# Autodesk Inventor assembly: Sample 1
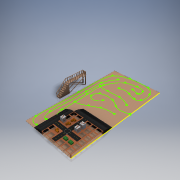
[picture p0: Inventor's stored thumbnail of the model, 180x180]
Saved by Autodesk Inventor 2019 (Build 230136000, 136)
## iProperties
Created: 2020-04-28
Part Number: Sample 1
Document SubType Name: Assembly
Designer: infinity
Author: infinity
## Documents named in this file (12)
- C:\Users\infinity\Documents\GitHub\barc_hardware\Track Sample 1\Sample 1.iam
- C:\Users\infinity\Documents\GitHub\barc_hardware\Track Sample 1\floor_50_100.ipt
- C:\Users\infinity\Documents\GitHub\barc_hardware\Track Sample 1\2ft stand.ipt
- C:\Users\infinity\Documents\GitHub\barc_hardware\Track Sample 1\Ramp 1.ipt
- C:\Users\infinity\Documents\GitHub\barc_hardware\Track Sample 1\driver stand.ipt
- C:\Users\infinity\Documents\GitHub\barc_hardware\Track Sample 1\house_1.ipt
- C:\Users\infinity\Documents\GitHub\barc_hardware\Track Sample 1\building_1.ipt
- C:\Users\infinity\Documents\GitHub\barc_hardware\Track Sample 1\apartment_1.ipt
- C:\Users\infinity\Documents\GitHub\barc_hardware\Track Sample 1\road_empty.ipt
- C:\Users\infinity\Documents\GitHub\barc_hardware\Track Sample 1\intersection_1.ipt
- C:\Users\infinity\Documents\GitHub\barc_hardware\Track Sample 1\black_mid_yellow line.ipt
- C:\Users\infinity\Documents\GitHub\barc_hardware\Track Sample 1\car110th.ipt
## Components (53 placed, 11 different names)
1. floor_50_100:1 — Mate:1, Mate:2, Mate:5, Flush:3, Flush:4, Mate:6, Flush:5
2. 2ft stand:1 — Mate:1, Mate:3, Flush:1, Mate:4, Flush:2, Flush:3, Flush:4, Flush:8, Mate:7, Mate:8, Mate:9, Mate:10, Mate:11, Mate:12, Mate:13, Mate:14, Flush:10, Mate:15, Mate:16, Mate:17, Mate:18, Flush:12, Mate:19, Mate:20, Mate:21, Flush:13, Mate:22, Flush:18, Mate:23, Mate:24, Mate:25, Mate:26, Mate:27, Mate:28, Mate:29, Mate:30, Mate:31, Mate:32, Mate:33, Mate:34, Mate:35, Mate:36, Mate:37, Flush:26, Mate:38, Mate:39, Flush:30, Mate:40, Mate:41, Mate:42, Mate:45, Mate:46, Mate:47, Mate:51, Mate:52, Mate:53
3. driver stand:1 — Mate:6, Flush:5
4. house_1:1 — Flush:6, Flush:7, Mate:7, Mate:8
5. house_1:2 — Flush:7, Flush:8, Mate:9, Mate:10, Flush:11
6. house_1:3 — Flush:6, Mate:11, Mate:12
7. building_1:1 — Mate:13, Mate:14, Flush:9, Flush:10, Flush:23
8. building_1:2 — Flush:9, Mate:15, Mate:16
9. apartment_1:1 — Mate:17, Mate:18, Flush:11
10. apartment_1:2 — Flush:12, Mate:19, Mate:20, Flush:25
11. apartment_1:3 — Mate:21, Flush:13, Mate:22
12. road_empty:1 — Flush:14, Flush:15, Flush:16, Flush:17, Flush:18, Mate:25, Mate:43
13. road_empty:2 — Mate:34, Mate:36, Flush:24, Flush:25, Mate:48
14. road_empty:3 — Flush:15, Flush:16, Mate:23, Mate:24, Mate:44
15. road_empty:4 — Flush:19, Flush:20, Mate:29
16. road_empty:5 — Flush:14, Flush:17, Mate:26, Flush:21, Mate:56, Tangent:1
17. road_empty:6 — Flush:19, Flush:20, Mate:27, Mate:28, Flush:21, Mate:50
18. road_empty:7 — Mate:30, Mate:33, Flush:22, Flush:23
19. road_empty:8 — Mate:31, Mate:32, Flush:22, Mate:54
20. road_empty:9 — Mate:35, Mate:37, Flush:24
21. intersection_1:1 — Flush:26, Mate:38, Mate:39, Mate:49, Mate:55
22. black_mid_yellow line:1 — Flush:27, Flush:30, Mate:40, Mate:41
23. black_mid_yellow line:2 — Flush:27, Mate:44, Mate:45
24. black_mid_yellow line:4 — Mate:42, Mate:43
25. black_mid_yellow line:5 — Flush:31, Flush:32, Flush:41, Flush:42, Flush:43, Flush:44, Mate:53, Mate:56
26. black_mid_yellow line:7 — Flush:33, Flush:35, Flush:37, Flush:38, Mate:47, Mate:49
27. black_mid_yellow line:8 — Flush:35, Flush:36, Flush:40, Mate:52
28. black_mid_yellow line:9 — Flush:33, Flush:34, Flush:39, Flush:40, Mate:51
29. black_mid_yellow line:10 — Flush:36, Flush:37, Mate:46, Mate:48
30. black_mid_yellow line:11 — Flush:34, Flush:38, Flush:39, Mate:50
31. black_mid_yellow line:12 — Flush:32, Flush:41, Flush:43, Mate:54, Mate:55
32. black_mid_yellow line:13 — Flush:31, Flush:42, Flush:44, Mate:57
33. car110th:1 — Tangent:1
34. Ramp 1:1 — Mate:2, Mate:3, Flush:1
35. Ramp 1:2
36. Ramp 1:3
37. Ramp 1:4
38. Ramp 1:5
39. Ramp 1:6 — Mate:57
40. Ramp 1:7
41. Ramp 1:8
42. Ramp 1:9
43. Ramp 1:10
44. Ramp 1:11 — Mate:4, Flush:2, Mate:5
45. Ramp 1:12
46. Ramp 1:13
47. Ramp 1:14
48. Ramp 1:15
49. Ramp 1:16
50. Ramp 1:17
51. Ramp 1:18
52. Ramp 1:19
53. Ramp 1:20
## Component patterns: (10 elements, first: Ramp 1:1), (10 elements, first: Ramp 1:11)
## Relationships (100: Mate 57, Flush 42, Tangent 1)
- Mate:1: floor_50_100:1 ↔ 2ft stand:1
- Mate:2: floor_50_100:1 ↔ Ramp 1:1
- Mate:3: 2ft stand:1 ↔ Ramp 1:1
- Flush:1: 2ft stand:1 ↔ Ramp 1:1
- Mate:4: 2ft stand:1 ↔ Ramp 1:11
- Flush:2: 2ft stand:1 ↔ Ramp 1:11
- Mate:5: floor_50_100:1 ↔ Ramp 1:11
- Flush:3: floor_50_100:1 ↔ 2ft stand:1
- Flush:4: floor_50_100:1 ↔ 2ft stand:1
- Mate:6 (914.4 mm): floor_50_100:1 ↔ driver stand:1
- Flush:5: floor_50_100:1 ↔ driver stand:1
- Flush:6: house_1:1 ↔ house_1:3
- Flush:7: house_1:1 ↔ house_1:2
- Flush:8: 2ft stand:1 ↔ house_1:2
- Mate:7: 2ft stand:1 ↔ house_1:1
- Mate:8: 2ft stand:1 ↔ house_1:1
- Mate:9: 2ft stand:1 ↔ house_1:2
- Mate:10: 2ft stand:1 ↔ house_1:2
- Mate:11: 2ft stand:1 ↔ house_1:3
- Mate:12: 2ft stand:1 ↔ house_1:3
- Mate:13: 2ft stand:1 ↔ building_1:1
- Mate:14: 2ft stand:1 ↔ building_1:1
- Flush:9: building_1:1 ↔ building_1:2
- Flush:10: 2ft stand:1 ↔ building_1:1
- Mate:15: 2ft stand:1 ↔ building_1:2
- Mate:16: 2ft stand:1 ↔ building_1:2
- Mate:17: 2ft stand:1 ↔ apartment_1:1
- Mate:18: 2ft stand:1 ↔ apartment_1:1
- Flush:11: house_1:2 ↔ apartment_1:1
- Flush:12: 2ft stand:1 ↔ apartment_1:2
- Mate:19: 2ft stand:1 ↔ apartment_1:2
- Mate:20: 2ft stand:1 ↔ apartment_1:2
- Mate:21: 2ft stand:1 ↔ apartment_1:3
- Flush:13: 2ft stand:1 ↔ apartment_1:3
- Mate:22: 2ft stand:1 ↔ apartment_1:3
- Flush:14: road_empty:1 ↔ road_empty:5
- Flush:15: road_empty:1 ↔ road_empty:3
- Flush:16: road_empty:1 ↔ road_empty:3
- Flush:17: road_empty:1 ↔ road_empty:5
- Flush:18: 2ft stand:1 ↔ road_empty:1
- Mate:23: 2ft stand:1 ↔ road_empty:3
- Mate:24: 2ft stand:1 ↔ road_empty:3
- Mate:25: 2ft stand:1 ↔ road_empty:1
- Mate:26: 2ft stand:1 ↔ road_empty:5
- Flush:19: road_empty:4 ↔ road_empty:6
- Flush:20: road_empty:4 ↔ road_empty:6
- Mate:27: 2ft stand:1 ↔ road_empty:6
- Mate:28: 2ft stand:1 ↔ road_empty:6
- Flush:21: road_empty:5 ↔ road_empty:6
- Mate:29: 2ft stand:1 ↔ road_empty:4
- Mate:30: 2ft stand:1 ↔ road_empty:7
- Mate:31: 2ft stand:1 ↔ road_empty:8
- Mate:32: 2ft stand:1 ↔ road_empty:8
- Mate:33: 2ft stand:1 ↔ road_empty:7
- Flush:22: road_empty:7 ↔ road_empty:8
- Flush:23: building_1:1 ↔ road_empty:7
- Mate:34: 2ft stand:1 ↔ road_empty:2
- Mate:35: 2ft stand:1 ↔ road_empty:9
- Mate:36: 2ft stand:1 ↔ road_empty:2
- Mate:37: 2ft stand:1 ↔ road_empty:9
- Flush:24: road_empty:2 ↔ road_empty:9
- Flush:25: apartment_1:2 ↔ road_empty:2
- Flush:26: 2ft stand:1 ↔ intersection_1:1
- Mate:38: 2ft stand:1 ↔ intersection_1:1
- Mate:39: 2ft stand:1 ↔ intersection_1:1
- Flush:27: black_mid_yellow line:1 ↔ black_mid_yellow line:2
- Flush:30: 2ft stand:1 ↔ black_mid_yellow line:1
- Mate:40: 2ft stand:1 ↔ black_mid_yellow line:1
- Mate:41: 2ft stand:1 ↔ black_mid_yellow line:1
- Mate:42: 2ft stand:1 ↔ black_mid_yellow line:4
- Mate:43: road_empty:1 ↔ black_mid_yellow line:4
- Mate:44: road_empty:3 ↔ black_mid_yellow line:2
- Mate:45: 2ft stand:1 ↔ black_mid_yellow line:2
- Flush:31: black_mid_yellow line:5 ↔ black_mid_yellow line:13
- Flush:32: black_mid_yellow line:5 ↔ black_mid_yellow line:12
- Flush:33: black_mid_yellow line:7 ↔ black_mid_yellow line:9
- Flush:34: black_mid_yellow line:9 ↔ black_mid_yellow line:11
- Flush:35: black_mid_yellow line:7 ↔ black_mid_yellow line:8
- Flush:36: black_mid_yellow line:8 ↔ black_mid_yellow line:10
- Flush:37: black_mid_yellow line:7 ↔ black_mid_yellow line:10
- Flush:38: black_mid_yellow line:7 ↔ black_mid_yellow line:11
- Flush:39: black_mid_yellow line:9 ↔ black_mid_yellow line:11
- Flush:40: black_mid_yellow line:8 ↔ black_mid_yellow line:9
- Mate:46: 2ft stand:1 ↔ black_mid_yellow line:10
- Mate:47: 2ft stand:1 ↔ black_mid_yellow line:7
- Mate:48: road_empty:2 ↔ black_mid_yellow line:10
- Mate:49: intersection_1:1 ↔ black_mid_yellow line:7
- Mate:50: road_empty:6 ↔ black_mid_yellow line:11
- Mate:51: 2ft stand:1 ↔ black_mid_yellow line:9
- Mate:52: 2ft stand:1 ↔ black_mid_yellow line:8
- Flush:41: black_mid_yellow line:5 ↔ black_mid_yellow line:12
- Flush:42: black_mid_yellow line:5 ↔ black_mid_yellow line:13
- Flush:43: black_mid_yellow line:5 ↔ black_mid_yellow line:12
- Flush:44: black_mid_yellow line:5 ↔ black_mid_yellow line:13
- Mate:53: 2ft stand:1 ↔ black_mid_yellow line:5
- Mate:54: road_empty:8 ↔ black_mid_yellow line:12
- Mate:55: intersection_1:1 ↔ black_mid_yellow line:12
- Mate:56: road_empty:5 ↔ black_mid_yellow line:5
- Mate:57: black_mid_yellow line:13 ↔ Ramp 1:6
- Tangent:1: road_empty:5 ↔ car110th:1
